# Autodesk Inventor assembly: z_carriage_assembly
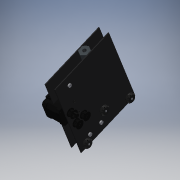
[picture p0: Inventor's stored thumbnail of the model, 180x180]
Saved by Autodesk Inventor 2018 (Build 220112000, 112)
## iProperties
Created: 2017-11-16
Part Number: z_carriage_assembly
Document SubType Name: Assembly
Designer: g
Author: g
## Documents named in this file (16)
- C:\Users\g\Desktop\AUG_inventor\z_carriage_assembly.iam
- C:\Users\g\Desktop\AUG_inventor\tieplate_big.ipt
- C:\Users\g\Desktop\AUG_inventor\M3 X 10mm Screw.ipt
- C:\Users\g\Desktop\AUG_inventor\NEMA17 w connector metric.ipt
- C:\Users\g\Desktop\AUG_inventor\GT2Pulley metric.ipt
- C:\Users\g\Desktop\AUG_inventor\GT2Bearing metric.ipt
- C:\Users\g\Desktop\AUG_inventor\M5 x 12mm Screw.ipt
- C:\Users\g\Desktop\AUG_inventor\m5x12mmscrew.ipt
- C:\Users\g\Desktop\AUG_inventor\5mmx20mmx8mm bearing.ipt
- C:\Users\g\Desktop\AUG_inventor\5mmx20mmx8mm bearing_MIR1.ipt
- C:\Users\g\Desktop\AUG_inventor\m5x12mmscrew_MIR1.ipt
- C:\Users\g\Desktop\AUG_inventor\5M nut 20mm_MIR.ipt
- C:\Users\g\Desktop\AUG_inventor\5mmx20mmx8mm bearing_MIR2_MIR.ipt
- C:\Users\g\Desktop\AUG_inventor\m5x12mmscrew_MIR2_MIR.ipt
- C:\Users\g\Desktop\AUG_inventor\5mmx20mmx8mm bearing_MIR3_MIR_MIR.ipt
- C:\Users\g\Desktop\AUG_inventor\m5x12mmscrew_MIR3_MIR_MIR.ipt
## Components (30 placed, 15 different names)
1. 5M nut 20mm_MIR:1 — Mate:320, Flush:182, Mate:321, Mate:322, Mate:323
2. 5M nut 20mm_MIR:2 — Mate:320
3. 5mmx20mmx8mm bearing_MIR2_MIR:2 — Cylindrical:136
4. m5x12mmscrew_MIR2_MIR:1 — Cylindrical:136
5. 5mmx20mmx8mm bearing_MIR3_MIR_MIR:1 — Cylindrical:139
6. 5mmx20mmx8mm bearing_MIR3_MIR_MIR:2 — Cylindrical:138
7. m5x12mmscrew_MIR3_MIR_MIR:1 — Cylindrical:138
8. m5x12mmscrew_MIR3_MIR_MIR:2 — Cylindrical:139
9. tieplate_big:2 — Flush:167, Flush:168, Mate:262, Mate:263, Mate:264, Cylindrical:113, Cylindrical:114, Cylindrical:115, Symmetry:3, Flush:179, Symmetry:4, Symmetry:5, Mate:321
10. tieplate_big:3 — Flush:167, Flush:168, Symmetry:3, Mate:265, Mate:266, Mate:267, Cylindrical:116, Cylindrical:117, Cylindrical:118, Mate:286, Flush:180, Mate:300, Mate:301, Mate:307, Mate:308, Mate:309, Mate:310, Flush:181, Mate:311, Mate:314, Mate:315, Symmetry:4, Symmetry:5, Flush:182, Mate:322, Mate:323
11. 5mmx20mmx8mm bearing:4 — Rotational:120
12. 5mmx20mmx8mm bearing:5 — Rotational:8
13. 5mmx20mmx8mm bearing:6 — Rotational:9
14. m5x12mmscrew:4 — Mate:264, Cylindrical:115, Rotational:8
15. m5x12mmscrew:5 — Mate:263, Cylindrical:114, Rotational:120
16. m5x12mmscrew:6 — Mate:262, Cylindrical:113, Rotational:9
17. 5mmx20mmx8mm bearing_MIR1:1 — Rotational:11
18. 5mmx20mmx8mm bearing_MIR1:2 — Rotational:10
19. 5mmx20mmx8mm bearing_MIR1:3 — Rotational:12
20. m5x12mmscrew_MIR1:1 — Rotational:10, Mate:267, Cylindrical:116
21. m5x12mmscrew_MIR1:2 — Rotational:11, Mate:266, Cylindrical:118
22. m5x12mmscrew_MIR1:3 — Rotational:12, Mate:265, Cylindrical:117
23. NEMA17 w connector metric:5 — Mate:286, Flush:179, Flush:180, Cylindrical:130, Cylindrical:131, Rigid:9
24. M3 X 10mm Screw:59 — Cylindrical:130, Mate:300
25. M3 X 10mm Screw:60 — Cylindrical:131, Mate:301
26. GT2Pulley metric:2 — Rigid:9
27. GT2Bearing metric:5 — Mate:308, Mate:309, Mate:310, Mate:316, Mate:317
28. GT2Bearing metric:6 — Mate:307, Flush:181, Mate:311, Mate:318, Mate:319
29. M5 x 12mm Screw:6 — Mate:315, Mate:318, Mate:319
30. M5 x 12mm Screw:7 — Mate:314, Mate:316, Mate:317
## Relationships (51: Mate 24, CylindricalJoint 11, Flush 6, RevoluteJoint 6, Symmetry 3, WeldJoint 1)
- Flush:167: tieplate_big:2 ↔ tieplate_big:3
- Flush:168: tieplate_big:2 ↔ tieplate_big:3
- Mate:262: tieplate_big:2 ↔ m5x12mmscrew:6
- Mate:263: tieplate_big:2 ↔ m5x12mmscrew:5
- Mate:264: tieplate_big:2 ↔ m5x12mmscrew:4
- Cylindrical:113: tieplate_big:2 ↔ m5x12mmscrew:6
- Cylindrical:114: tieplate_big:2 ↔ m5x12mmscrew:5
- Cylindrical:115: tieplate_big:2 ↔ m5x12mmscrew:4
- Rotational:120 [RevoluteJoint] (-0.5 mm): 5mmx20mmx8mm bearing:4 ↔ m5x12mmscrew:5
- Rotational:8 [RevoluteJoint] (-0.5 mm): 5mmx20mmx8mm bearing:5 ↔ m5x12mmscrew:4
- Rotational:9 [RevoluteJoint] (-0.5 mm): 5mmx20mmx8mm bearing:6 ↔ m5x12mmscrew:6
- Symmetry:3: tieplate_big:2 ↔ tieplate_big:3
- Rotational:10 [RevoluteJoint] (-0.5 mm): 5mmx20mmx8mm bearing_MIR1:2 ↔ m5x12mmscrew_MIR1:1
- Rotational:11 [RevoluteJoint] (-0.5 mm): 5mmx20mmx8mm bearing_MIR1:1 ↔ m5x12mmscrew_MIR1:2
- Rotational:12 [RevoluteJoint] (0.5 mm): 5mmx20mmx8mm bearing_MIR1:3 ↔ m5x12mmscrew_MIR1:3
- Mate:265: tieplate_big:3 ↔ m5x12mmscrew_MIR1:3
- Mate:266: tieplate_big:3 ↔ m5x12mmscrew_MIR1:2
- Mate:267: tieplate_big:3 ↔ m5x12mmscrew_MIR1:1
- Cylindrical:116: tieplate_big:3 ↔ m5x12mmscrew_MIR1:1
- Cylindrical:117: tieplate_big:3 ↔ m5x12mmscrew_MIR1:3
- Cylindrical:118: tieplate_big:3 ↔ m5x12mmscrew_MIR1:2
- Mate:286 (1.5 mm): tieplate_big:3 ↔ NEMA17 w connector metric:5
- Flush:179 (-10 mm): tieplate_big:2 ↔ NEMA17 w connector metric:5
- Flush:180 (55 mm): tieplate_big:3 ↔ NEMA17 w connector metric:5
- Cylindrical:130: NEMA17 w connector metric:5 ↔ M3 X 10mm Screw:59
- Cylindrical:131: NEMA17 w connector metric:5 ↔ M3 X 10mm Screw:60
- Rigid:9 [WeldJoint]: NEMA17 w connector metric:5 ↔ GT2Pulley metric:2
- Mate:300: tieplate_big:3 ↔ M3 X 10mm Screw:59
- Mate:301: tieplate_big:3 ↔ M3 X 10mm Screw:60
- Mate:307: tieplate_big:3 ↔ GT2Bearing metric:6
- Mate:308: tieplate_big:3 ↔ GT2Bearing metric:5
- Mate:309 (-5 mm): tieplate_big:3 ↔ GT2Bearing metric:5
- Mate:310 (-100 mm): tieplate_big:3 ↔ GT2Bearing metric:5
- Flush:181 (25 mm): tieplate_big:3 ↔ GT2Bearing metric:6
- Mate:311 (-99 mm): tieplate_big:3 ↔ GT2Bearing metric:6
- Mate:314: tieplate_big:3 ↔ M5 x 12mm Screw:7
- Mate:315: tieplate_big:3 ↔ M5 x 12mm Screw:6
- Mate:316: GT2Bearing metric:5 ↔ M5 x 12mm Screw:7
- Mate:317: GT2Bearing metric:5 ↔ M5 x 12mm Screw:7
- Mate:318: GT2Bearing metric:6 ↔ M5 x 12mm Screw:6
- Mate:319: GT2Bearing metric:6 ↔ M5 x 12mm Screw:6
- Symmetry:4: tieplate_big:2 ↔ tieplate_big:3
- Mate:320: 5M nut 20mm_MIR:1 ↔ 5M nut 20mm_MIR:2
- Symmetry:5: tieplate_big:2 ↔ tieplate_big:3
- Cylindrical:136: 5mmx20mmx8mm bearing_MIR2_MIR:2 ↔ m5x12mmscrew_MIR2_MIR:1
- Cylindrical:138: 5mmx20mmx8mm bearing_MIR3_MIR_MIR:2 ↔ m5x12mmscrew_MIR3_MIR_MIR:1
- Cylindrical:139: 5mmx20mmx8mm bearing_MIR3_MIR_MIR:1 ↔ m5x12mmscrew_MIR3_MIR_MIR:2
- Flush:182: 5M nut 20mm_MIR:1 ↔ tieplate_big:3
- Mate:321: 5M nut 20mm_MIR:1 ↔ tieplate_big:2
- Mate:322 (-40 mm): 5M nut 20mm_MIR:1 ↔ tieplate_big:3
- Mate:323: 5M nut 20mm_MIR:1 ↔ tieplate_big:3
